# Autodesk Inventor assembly: omni_platformaV2
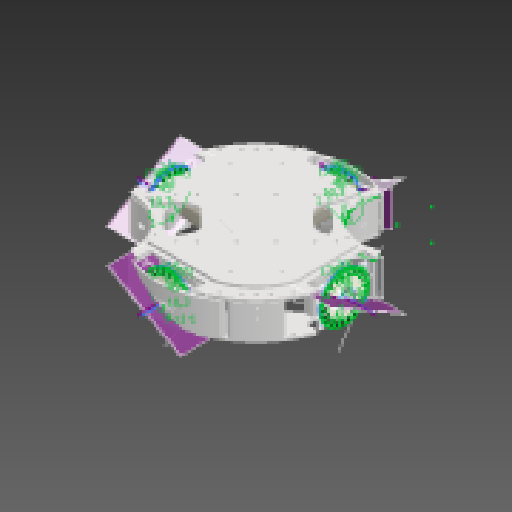
[picture p0: Inventor's stored thumbnail of the model, 512x512]
Saved by Autodesk Inventor 2023 (Build 270158000, 158)
## iProperties
Created: 2025-08-05
Part Number: omni_platformaV2
Document SubType Name: Assembly
Designer: daa
Author: daa
## Documents named in this file (12)
- C:\Users\daa\Documents\DASH_V2\omni_platforma\omni_platformaV2.iam
- C:\Users\daa\Documents\DASH_V2\omni_platforma\bottom.ipt
- C:\Users\daa\Documents\DASH_V2\omni_platforma\top_v2.ipt
- C:\Users\daa\Documents\DASH_V2\omni_platforma\dribler_ball.ipt
- C:\Users\daa\Documents\DASH_V2\omni_platforma\Деталь1.ipt
- C:\Users\daa\Documents\DASH_V2\omni_platforma\fastenin_motor.ipt
- C:\Users\daa\Documents\DASH_V2\omni_platforma\motor20.ipt
- C:\Users\daa\Documents\DASH_V2\omni_platforma\handle mount.ipt
- C:\Users\daa\Documents\DASH_V2\omni_platforma\protect.ipt
- C:\Users\daa\Documents\DASH_V2\omni_platforma\Wheel.iam
- C:\Users\daa\Documents\DASH_V2\omni_platforma\Solenoid.iam
- C:\Users\daa\Documents\DASH_V2\omni_platforma\plata_v2.ipt
## Components (22 placed, 11 different names)
1. bottom:1 — Совмещение:1, Совмещение:2, Совмещение:3, Совмещение:4, Совмещение:5, Совмещение:6, Совмещение:7, Совмещение:8, Совмещение:9, Совмещение:10, Совмещение:11, Совмещение:12, Совмещение:13, Совмещение:14, Совмещение:15, Совмещение:16, С поворотом:5, С поворотом:6, С поворотом:7
2. dribler_ball:1 — Совмещение:1, Совмещение:2
3. Деталь1:1 — Совмещение:3, Совмещение:4, Совмещение:17
4. fastenin_motor:1 — Совмещение:5, Совмещение:6, Жесткий:4
5. fastenin_motor:2 — Совмещение:11, Совмещение:12, Жесткий:1
6. fastenin_motor:3 — Совмещение:7, Совмещение:8, Жесткий:3
7. fastenin_motor:4 — Совмещение:9, Совмещение:10, Жесткий:2
8. motor20:1 — Жесткий:1, С поворотом:4
9. motor20:2 — Жесткий:2, С поворотом:2
10. motor20:3 — Жесткий:3, С поворотом:1
11. motor20:4 — Жесткий:4, С поворотом:3
12. handle mount:1 — Совмещение:13, Совмещение:14
13. handle mount:2 — Совмещение:15, Совмещение:16
14. protect:1 — С поворотом:6
15. protect:2 — С поворотом:5
16. Wheel:1 [sub-assembly] — С поворотом:1
17. Wheel:2 [sub-assembly] — С поворотом:2
18. Wheel:3 [sub-assembly] — С поворотом:3
19. Wheel:4 [sub-assembly] — С поворотом:4
20. Solenoid:1 [sub-assembly] — С поворотом:7
21. top_v2:1 — Совмещение:17, Совмещение:18
22. plata_v2:1 — Совмещение:18
## Relationships (29: Mate 18, RevoluteJoint 7, WeldJoint 4)
- Совмещение:1 [Mate]: bottom:1 ↔ dribler_ball:1
- Совмещение:2 [Mate]: bottom:1 ↔ dribler_ball:1
- Совмещение:3 [Mate]: bottom:1 ↔ Деталь1:1
- Совмещение:4 [Mate]: bottom:1 ↔ Деталь1:1
- Совмещение:5 [Mate]: bottom:1 ↔ fastenin_motor:1
- Совмещение:6 [Mate]: bottom:1 ↔ fastenin_motor:1
- Совмещение:7 [Mate]: bottom:1 ↔ fastenin_motor:3
- Совмещение:8 [Mate]: bottom:1 ↔ fastenin_motor:3
- Совмещение:9 [Mate]: bottom:1 ↔ fastenin_motor:4
- Совмещение:10 [Mate]: bottom:1 ↔ fastenin_motor:4
- Совмещение:11 [Mate]: bottom:1 ↔ fastenin_motor:2
- Совмещение:12 [Mate]: bottom:1 ↔ fastenin_motor:2
- Жесткий:1 [WeldJoint] (-5 mm): fastenin_motor:2 ↔ motor20:1
- Жесткий:2 [WeldJoint] (-5 mm): fastenin_motor:4 ↔ motor20:2
- Жесткий:3 [WeldJoint] (-5 mm): fastenin_motor:3 ↔ motor20:3
- Жесткий:4 [WeldJoint] (-5 mm): fastenin_motor:1 ↔ motor20:4
- Совмещение:13 [Mate]: bottom:1 ↔ handle mount:1
- Совмещение:14 [Mate]: bottom:1 ↔ handle mount:1
- Совмещение:15 [Mate]: bottom:1 ↔ handle mount:2
- Совмещение:16 [Mate]: bottom:1 ↔ handle mount:2
- С поворотом:1 [RevoluteJoint] (-4 mm): motor20:3 ↔ Wheel:1
- С поворотом:2 [RevoluteJoint] (-4 mm): motor20:2 ↔ Wheel:2
- С поворотом:3 [RevoluteJoint] (-4 mm): motor20:4 ↔ Wheel:3
- С поворотом:4 [RevoluteJoint] (-4 mm): motor20:1 ↔ Wheel:4
- С поворотом:5 [RevoluteJoint]: bottom:1 ↔ protect:2
- С поворотом:6 [RevoluteJoint]: bottom:1 ↔ protect:1
- С поворотом:7 [RevoluteJoint]: bottom:1 ↔ Solenoid:1
- Совмещение:17 [Mate]: Деталь1:1 ↔ top_v2:1
- Совмещение:18 [Mate]: top_v2:1 ↔ plata_v2:1
